# Autodesk Inventor assembly: front_right
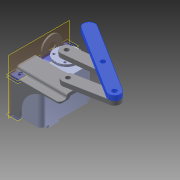
[picture p0: Inventor's stored thumbnail of the model, 180x180]
Saved by Autodesk Inventor 2014 (Build 180170000, 170)
## iProperties
Created: 2015-03-09
Part Number: front_right
Document SubType Name: Assembly
Designer: Hideyuki Takei
Author: Hideyuki Takei
## Documents named in this file (7)
- C:\Users\hide\Desktop\soth-bonsai\cad\front_right.iam
- C:\Users\hide\Desktop\soth-bonsai\cad\RS304MD_ServoHorn.ipt
- C:\Users\hide\Desktop\soth-bonsai\cad\RS304md-simple.ipt
- C:\Users\hide\Desktop\soth-bonsai\cad\servo-holder.ipt
- C:\Users\hide\Desktop\soth-bonsai\cad\link_long.ipt
- C:\Users\hide\Desktop\soth-bonsai\cad\link_short.ipt
- C:\Users\hide\Desktop\soth-bonsai\cad\leg.ipt
## Components (6 placed, 6 different names)
1. RS304MD_ServoHorn:1 — メイト:2, メイト:3, メイト:11
2. RS304md-simple:1 — メイト:2, メイト:3, メイト:4, メイト:5, メイト:6, メイト:10
3. servo-holder:1 — メイト:4, メイト:5, メイト:6, メイト:7, メイト:9, メイト:16, メイト:17
4. link_long:1 — メイト:7, メイト:9, メイト:12, メイト:13
5. link_short:1 — メイト:10, メイト:11, メイト:14, メイト:15
6. leg:1 — メイト:12, メイト:13, メイト:14, メイト:15
## Relationships (15: Mate 15)
- メイト:2 [Mate]: RS304MD_ServoHorn:1 ↔ RS304md-simple:1
- メイト:3 [Mate]: RS304MD_ServoHorn:1 ↔ RS304md-simple:1
- メイト:4 [Mate]: RS304md-simple:1 ↔ servo-holder:1
- メイト:5 [Mate]: RS304md-simple:1 ↔ servo-holder:1
- メイト:6 [Mate]: RS304md-simple:1 ↔ servo-holder:1
- メイト:7 [Mate]: servo-holder:1 ↔ link_long:1
- メイト:9 [Mate]: servo-holder:1 ↔ link_long:1
- メイト:10 [Mate]: RS304md-simple:1 ↔ link_short:1
- メイト:11 [Mate]: RS304MD_ServoHorn:1 ↔ link_short:1
- メイト:12 [Mate]: link_long:1 ↔ leg:1
- メイト:13 [Mate]: link_long:1 ↔ leg:1
- メイト:14 [Mate]: link_short:1 ↔ leg:1
- メイト:15 [Mate]: link_short:1 ↔ leg:1
- メイト:16 [Mate]: servo-holder:1
- メイト:17 [Mate]: servo-holder:1
